# Autodesk Inventor assembly: Frame 1780692296746
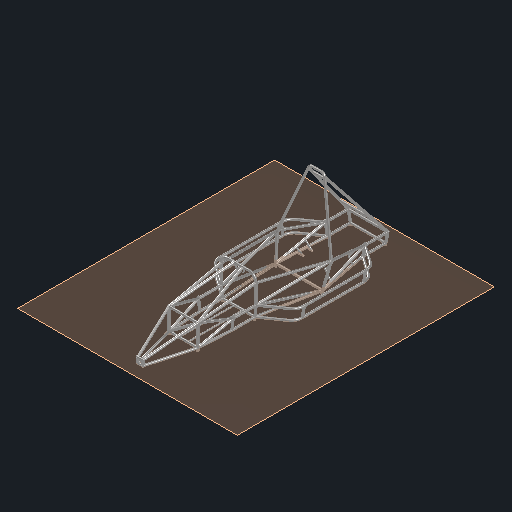
[picture p0: Inventor's stored thumbnail of the model, 512x512]
Saved by Autodesk Inventor 2026.2 (Build 302298010, 298A)
## iProperties
_FrameDoc: Frame Assembly
_Version: 25.0.0
Created: 2026-06-05
Part Number: Frame 1780692296746
Document SubType Name: Assembly
Designer: tasle
Mass: 133713 g
Surface Area: 77277.6 cm^2
Volume: 17033.5 cm^3
Density: 7.85 g/cm^3
Author: tasle
## Documents named in this file (83)
- C:\Users\tasle\Documents\PersonalProjects\FSAE\GOGO_FSAE_CAD\FrameV2\Frame\Frame 1780692296746.iam
- C:\Users\tasle\Documents\PersonalProjects\FSAE\GOGO_FSAE_CAD\FrameV2\Frame\Skeleton 1780692296747.ipt
- C:\Users\tasle\Documents\PersonalProjects\FSAE\GOGO_FSAE_CAD\FrameV2\Frame\ANSI 1 x 0.179 1780692302546.ipt
- C:\Users\tasle\Documents\PersonalProjects\FSAE\GOGO_FSAE_CAD\FrameV2\Frame\ANSI 1 x 0.179 1780692302574.ipt
- C:\Users\tasle\Documents\PersonalProjects\FSAE\GOGO_FSAE_CAD\FrameV2\Frame\ANSI 1 x 0.179 1780692302595.ipt
- C:\Users\tasle\Documents\PersonalProjects\FSAE\GOGO_FSAE_CAD\FrameV2\Frame\ANSI 1 x 0.179 1780692302622.ipt
- C:\Users\tasle\Documents\PersonalProjects\FSAE\GOGO_FSAE_CAD\FrameV2\Frame\ANSI 1 x 0.179 1780692302650.ipt
- C:\Users\tasle\Documents\PersonalProjects\FSAE\GOGO_FSAE_CAD\FrameV2\Frame\ANSI 1 x 0.179 1780692302672.ipt
- C:\Users\tasle\Documents\PersonalProjects\FSAE\GOGO_FSAE_CAD\FrameV2\Frame\ANSI 1 x 0.179 1780692302694.ipt
- C:\Users\tasle\Documents\PersonalProjects\FSAE\GOGO_FSAE_CAD\FrameV2\Frame\ANSI 1 x 0.179 1780692302716.ipt
- C:\Users\tasle\Documents\PersonalProjects\FSAE\GOGO_FSAE_CAD\FrameV2\Frame\ANSI 1 x 0.179 1780692302739.ipt
- C:\Users\tasle\Documents\PersonalProjects\FSAE\GOGO_FSAE_CAD\FrameV2\Frame\ANSI 1 x 0.179 1780692302759.ipt
- C:\Users\tasle\Documents\PersonalProjects\FSAE\GOGO_FSAE_CAD\FrameV2\Frame\ANSI 1 x 0.179 1780692302779.ipt
- C:\Users\tasle\Documents\PersonalProjects\FSAE\GOGO_FSAE_CAD\FrameV2\Frame\ANSI 1 x 0.179 1780692302799.ipt
- C:\Users\tasle\Documents\PersonalProjects\FSAE\GOGO_FSAE_CAD\FrameV2\Frame\ANSI 1 x 0.179 1780692302820.ipt
- C:\Users\tasle\Documents\PersonalProjects\FSAE\GOGO_FSAE_CAD\FrameV2\Frame\ANSI 1 x 0.179 1780692302840.ipt
- C:\Users\tasle\Documents\PersonalProjects\FSAE\GOGO_FSAE_CAD\FrameV2\Frame\ANSI 1 x 0.179 1780692302880.ipt
- C:\Users\tasle\Documents\PersonalProjects\FSAE\GOGO_FSAE_CAD\FrameV2\Frame\ANSI 1 x 0.179 1780692302901.ipt
- C:\Users\tasle\Documents\PersonalProjects\FSAE\GOGO_FSAE_CAD\FrameV2\Frame\ANSI 1 x 0.179 1780692302942.ipt
- C:\Users\tasle\Documents\PersonalProjects\FSAE\GOGO_FSAE_CAD\FrameV2\Frame\ANSI 1 x 0.179 1780692302962.ipt
- C:\Users\tasle\Documents\PersonalProjects\FSAE\GOGO_FSAE_CAD\FrameV2\Frame\ANSI 1 x 0.179 1780692302983.ipt
- C:\Users\tasle\Documents\PersonalProjects\FSAE\GOGO_FSAE_CAD\FrameV2\Frame\ANSI 1 x 0.179 1780692303004.ipt
- C:\Users\tasle\Documents\PersonalProjects\FSAE\GOGO_FSAE_CAD\FrameV2\Frame\ANSI 1 x 0.179 1780692303025.ipt
- C:\Users\tasle\Documents\PersonalProjects\FSAE\GOGO_FSAE_CAD\FrameV2\Frame\ANSI 1 x 0.179 1780692303065.ipt
- C:\Users\tasle\Documents\PersonalProjects\FSAE\GOGO_FSAE_CAD\FrameV2\Frame\ANSI 1 x 0.179 1780692303109.ipt
- C:\Users\tasle\Documents\PersonalProjects\FSAE\GOGO_FSAE_CAD\FrameV2\Frame\ANSI 1 x 0.179 1780692303131.ipt
- C:\Users\tasle\Documents\PersonalProjects\FSAE\GOGO_FSAE_CAD\FrameV2\Frame\ANSI 1 x 0.179 1780692303282.ipt
- C:\Users\tasle\Documents\PersonalProjects\FSAE\GOGO_FSAE_CAD\FrameV2\Frame\ANSI 1 x 0.179 1780692303302.ipt
- C:\Users\tasle\Documents\PersonalProjects\FSAE\GOGO_FSAE_CAD\FrameV2\Frame\ANSI 1 x 0.179 1780692303344.ipt
- C:\Users\tasle\Documents\PersonalProjects\FSAE\GOGO_FSAE_CAD\FrameV2\Frame\ANSI 1 x 0.179 1780692303426.ipt
- C:\Users\tasle\Documents\PersonalProjects\FSAE\GOGO_FSAE_CAD\FrameV2\Frame\ANSI 1 x 0.179 1780692303471.ipt
- C:\Users\tasle\Documents\PersonalProjects\FSAE\GOGO_FSAE_CAD\FrameV2\Frame\ANSI 1 x 0.179 1780692303492.ipt
- C:\Users\tasle\Documents\PersonalProjects\FSAE\GOGO_FSAE_CAD\FrameV2\Frame\ANSI 1 x 0.179 1780692303687.ipt
- C:\Users\tasle\Documents\PersonalProjects\FSAE\GOGO_FSAE_CAD\FrameV2\Frame\ANSI 1 x 0.179 1780692303707.ipt
- C:\Users\tasle\Documents\PersonalProjects\FSAE\GOGO_FSAE_CAD\FrameV2\Frame\ANSI 1 x 0.179 1780692303816.ipt
- C:\Users\tasle\Documents\PersonalProjects\FSAE\GOGO_FSAE_CAD\FrameV2\Frame\ANSI 1 x 0.179 1780692303838.ipt
- C:\Users\tasle\Documents\PersonalProjects\FSAE\GOGO_FSAE_CAD\FrameV2\Frame\ANSI 1 x 0.179 1780692303858.ipt
- C:\Users\tasle\Documents\PersonalProjects\FSAE\GOGO_FSAE_CAD\FrameV2\Frame\ANSI 1 x 0.179 1780692303879.ipt
- C:\Users\tasle\Documents\PersonalProjects\FSAE\GOGO_FSAE_CAD\FrameV2\Frame\ANSI 1 x 0.179 1780692303920.ipt
- C:\Users\tasle\Documents\PersonalProjects\FSAE\GOGO_FSAE_CAD\FrameV2\Frame\ANSI 1 x 0.179 1780692303940.ipt
- C:\Users\tasle\Documents\PersonalProjects\FSAE\GOGO_FSAE_CAD\FrameV2\Frame\ANSI 1 x 0.179 1780692303966.ipt
- C:\Users\tasle\Documents\PersonalProjects\FSAE\GOGO_FSAE_CAD\FrameV2\Frame\ANSI 1 x 0.179 1780692304008.ipt
- C:\Users\tasle\Documents\PersonalProjects\FSAE\GOGO_FSAE_CAD\FrameV2\Frame\ANSI 1 x 0.179 1780692304091.ipt
- C:\Users\tasle\Documents\PersonalProjects\FSAE\GOGO_FSAE_CAD\FrameV2\Frame\ANSI 1 x 0.179 1780692304111.ipt
- C:\Users\tasle\Documents\PersonalProjects\FSAE\GOGO_FSAE_CAD\FrameV2\Frame\ANSI 1 x 0.179 1780692304131.ipt
- C:\Users\tasle\Documents\PersonalProjects\FSAE\GOGO_FSAE_CAD\FrameV2\Frame\ANSI 1 x 0.179 1780692304151.ipt
- C:\Users\tasle\Documents\PersonalProjects\FSAE\GOGO_FSAE_CAD\FrameV2\Frame\ANSI 1 x 0.179 1780692304297.ipt
- C:\Users\tasle\Documents\PersonalProjects\FSAE\GOGO_FSAE_CAD\FrameV2\Frame\ANSI 1 x 0.179 1780692304340.ipt
- C:\Users\tasle\Documents\PersonalProjects\FSAE\GOGO_FSAE_CAD\FrameV2\Frame\ANSI 1 x 0.179 1780692304362.ipt
- C:\Users\tasle\Documents\PersonalProjects\FSAE\GOGO_FSAE_CAD\FrameV2\Frame\ANSI 1 x 0.179 1780692304384.ipt
- C:\Users\tasle\Documents\PersonalProjects\FSAE\GOGO_FSAE_CAD\FrameV2\Frame\ANSI 1 x 0.179 1780692304405.ipt
- C:\Users\tasle\Documents\PersonalProjects\FSAE\GOGO_FSAE_CAD\FrameV2\Frame\ANSI 1 x 0.179 1780692304425.ipt
- C:\Users\tasle\Documents\PersonalProjects\FSAE\GOGO_FSAE_CAD\FrameV2\Frame\ANSI 1 x 0.179 1780692304445.ipt
- C:\Users\tasle\Documents\PersonalProjects\FSAE\GOGO_FSAE_CAD\FrameV2\Frame\ANSI 1 x 0.179 1780692304465.ipt
- C:\Users\tasle\Documents\PersonalProjects\FSAE\GOGO_FSAE_CAD\FrameV2\Frame\ANSI 1 x 0.179 1780692304485.ipt
- C:\Users\tasle\Documents\PersonalProjects\FSAE\GOGO_FSAE_CAD\FrameV2\Frame\ANSI 1 x 0.179 1780692304506.ipt
- C:\Users\tasle\Documents\PersonalProjects\FSAE\GOGO_FSAE_CAD\FrameV2\Frame\ANSI 1 x 0.179 1780692304526.ipt
- C:\Users\tasle\Documents\PersonalProjects\FSAE\GOGO_FSAE_CAD\FrameV2\Frame\ANSI 1 x 0.179 1780692304546.ipt
- C:\Users\tasle\Documents\PersonalProjects\FSAE\GOGO_FSAE_CAD\FrameV2\Frame\ANSI 1 x 0.179 1780692304587.ipt
- C:\Users\tasle\Documents\PersonalProjects\FSAE\GOGO_FSAE_CAD\FrameV2\Frame\ANSI 1 x 0.179 1782332076807.ipt
- C:\Users\tasle\Documents\PersonalProjects\FSAE\GOGO_FSAE_CAD\FrameV2\Frame\ANSI 1 x 0.179 1782332200115.ipt
- C:\Users\tasle\Documents\PersonalProjects\FSAE\GOGO_FSAE_CAD\FrameV2\Frame\ANSI 1 x 0.179 1782332294883.ipt
- C:\Users\tasle\Documents\PersonalProjects\FSAE\GOGO_FSAE_CAD\FrameV2\Frame\ANSI 1 x 0.179 1782332350122.ipt
- C:\Users\tasle\Documents\PersonalProjects\FSAE\GOGO_FSAE_CAD\FrameV2\Frame\ANSI 1 x 0.179 1782332425793.ipt
- C:\Users\tasle\Documents\PersonalProjects\FSAE\GOGO_FSAE_CAD\FrameV2\Frame\ANSI 1 x 0.179 1782332467531.ipt
- C:\Users\tasle\Documents\PersonalProjects\FSAE\GOGO_FSAE_CAD\FrameV2\Frame\ANSI 1 x 0.179 1782334188549.ipt
- C:\Users\tasle\Documents\PersonalProjects\FSAE\GOGO_FSAE_CAD\FrameV2\Frame\ANSI 1 x 0.179 1782334250193.ipt
- C:\Users\tasle\Documents\PersonalProjects\FSAE\GOGO_FSAE_CAD\FrameV2\Frame\ANSI 1_2 x 0.109 1783344969371.ipt
- C:\Users\tasle\Documents\PersonalProjects\FSAE\GOGO_FSAE_CAD\FrameV2\Frame\ANSI 1_2 x 0.109 1783344969395.ipt
- C:\Users\tasle\Documents\PersonalProjects\FSAE\GOGO_FSAE_CAD\FrameV2\Frame\ANSI 1_2 x 0.109 1783352366176.ipt
- C:\Users\tasle\Documents\PersonalProjects\FSAE\GOGO_FSAE_CAD\FrameV2\Frame\ANSI 1_2 x 0.109 1783352366199.ipt
- C:\Users\tasle\Documents\PersonalProjects\FSAE\GOGO_FSAE_CAD\Frame Assembly\FrameV2\Frame\ANSI 1_2 x 0.109 1785174968284.ipt
- C:\Users\tasle\Documents\PersonalProjects\FSAE\GOGO_FSAE_CAD\Frame Assembly\FrameV2\Frame\ANSI 1_2 x 0.109 1785174968323.ipt
- C:\Users\tasle\Documents\PersonalProjects\FSAE\GOGO_FSAE_CAD\Frame Assembly\FrameV2\Frame\ANSI 1_2 x 0.109 1785174968359.ipt
- C:\Users\tasle\Documents\PersonalProjects\FSAE\GOGO_FSAE_CAD\Frame Assembly\FrameV2\Frame\ANSI 1_2 x 0.109 1785177095365.ipt
- C:\Users\tasle\Documents\PersonalProjects\FSAE\GOGO_FSAE_CAD\Frame Assembly\FrameV2\Frame\ANSI 1_2 x 0.109 1785177095400.ipt
- C:\Users\tasle\Documents\PersonalProjects\FSAE\GOGO_FSAE_CAD\Frame Assembly\FrameV2\Frame\ANSI 1_2 x 0.109 1785177095431.ipt
- C:\Users\tasle\Documents\PersonalProjects\FSAE\GOGO_FSAE_CAD\Frame Assembly\FrameV2\Frame\ANSI 1_2 x 0.109 1785264200197.ipt
- C:\Users\tasle\Documents\PersonalProjects\FSAE\GOGO_FSAE_CAD\Frame Assembly\FrameV2\Frame\ANSI 1_2 x 0.109 1785264200234.ipt
- C:\Users\tasle\Documents\PersonalProjects\FSAE\GOGO_FSAE_CAD\Frame Assembly\FrameV2\Frame\ANSI 1_2 x 0.109 1785264200274.ipt
- C:\Users\tasle\Documents\PersonalProjects\FSAE\GOGO_FSAE_CAD\Frame Assembly\FrameV2\Frame\ANSI 1_2 x 0.109 1785264200308.ipt
- C:\Users\tasle\Documents\PersonalProjects\FSAE\GOGO_FSAE_CAD\Frame Assembly\FrameV2\Frame\ANSI 1 x 0.133 1785638103512.ipt
- C:\Users\tasle\Documents\PersonalProjects\FSAE\GOGO_FSAE_CAD\Frame Assembly\FrameV2\Frame\ANSI 1 x 0.133 1785638103546.ipt
## Components (82 placed, 46 different names)
1. Reference Skeleton
2. ANSI 1 x 0.179 - 26.119:1
3. ANSI 1 x 0.179 - 24.499:1
4. ANSI 1 x 0.179 - 26.119:2
5. ANSI 1 x 0.179 - 24.499:2
6. ANSI 1 x 0.179 - 4.076:1
7. ANSI 1 x 0.179 - 4.076:2
8. ANSI 1 x 0.179 - 4.076:3
9. ANSI 1 x 0.179 - 4.076:4
10. ANSI 1 x 0.179 - 15.748:1
11. ANSI 1 x 0.179 - 19.685:1
12. ANSI 1 x 0.179 - 13.971:1
13. ANSI 1 x 0.179 - 17.068:2
14. ANSI 1 x 0.179 - 13.971:2
15. ANSI 1 x 0.179 - 18.741:1
16. ANSI 1 x 0.179 - 18.741:2
17. ANSI 1 x 0.179 - 18.741:3
18. ANSI 1 x 0.179 - 6.935:1
19. ANSI 1 x 0.179 - 18.741:4
20. ANSI 1 x 0.179 - 32.006:1
21. ANSI 1 x 0.179 - 30.721:1
22. ANSI 1 x 0.179 - 30.721:2
23. ANSI 1 x 0.179 - 12.598:4
24. ANSI 1 x 0.179 - 6.935:3
25. ANSI 1 x 0.179 - 12.598:5
26. ANSI 1 x 0.179 - 17.717:1
27. ANSI 1 x 0.179 - 36.643:1
28. ANSI 1 x 0.179 - 36.727:1
29. ANSI 1 x 0.179 - 34.146:1
30. ANSI 1 x 0.179 - 33.363:1
31. ANSI 1 x 0.179 - 5.975:5
32. ANSI 1 x 0.179 - 5.975:6
33. ANSI 1 x 0.179 - 5.975:7
34. ANSI 1 x 0.179 - 36.643:2
35. ANSI 1 x 0.179 - 36.727:2
36. ANSI 1 x 0.179 - 34.146:2
37. ANSI 1 x 0.179 - 33.363:2
38. ANSI 1 x 0.179 - 26.472:1
39. ANSI 1 x 0.179 - 25.469:1
40. ANSI 1 x 0.179 - 23.324:1
41. ANSI 1 x 0.179 - 5.975:8
42. ANSI 1 x 0.179 - 8.022:9
43. ANSI 1 x 0.179 - 8.022:10
44. ANSI 1 x 0.179 - 26.472:2
45. ANSI 1 x 0.179 - 23.324:2
46. ANSI 1 x 0.179 - 47.004:1
47. ANSI 1 x 0.179 - 47.004:2
48. ANSI 1 x 0.179 - 12.598:8
49. ANSI 1 x 0.179 - 25.469:2
50. ANSI 1 x 0.179 - 25.591:1
51. ANSI 1 x 0.179 - 12.598:9
52. ANSI 1 x 0.179 - 7.828:11
53. ANSI 1 x 0.179 - 19.291:2
54. ANSI 1 x 0.179 - 23.264:2
55. ANSI 1 x 0.179 - 12.598:10
56. ANSI 1 x 0.179 - 12.598:11
57. ANSI 1 x 0.179 - 7.828:12
58. ANSI 1 x 0.179 - 32.006:1
59. ANSI 1 x 0.179 - 108.156:1
60. ANSI 1 x 0.179 - 59.522:1
61. ANSI 1 x 0.179 - 70.709:1
62. ANSI 1 x 0.179 - 70.709:2
63. ANSI 1 x 0.179 - 70.709:3
64. ANSI 1 x 0.179 - 70.709:4
65. ANSI 1 x 0.179 - 30.342:1
66. ANSI 1 x 0.179 - 30.342:2
67. ANSI 1/2 x 0.109 - 29.297:1
68. ANSI 1/2 x 0.109 - 29.297:2
69. ANSI 1/2 x 0.109 - 3.643:1
70. ANSI 1/2 x 0.109 - 3.643:2
71. ANSI 1/2 x 0.109 - 9.374:1
72. ANSI 1/2 x 0.109 - 5.512:1
73. ANSI 1/2 x 0.109 - 0.984:1
74. ANSI 1/2 x 0.109 - 5.653:1
75. ANSI 1/2 x 0.109 - 0.787:1
76. ANSI 1/2 x 0.109 - 3.985:1
77. ANSI 1/2 x 0.109 - 4.983:1
78. ANSI 1/2 x 0.109 - 3.937:1
79. ANSI 1/2 x 0.109 - 5.549:1
80. ANSI 1/2 x 0.109 - 3.355:1
81. ANSI 1 x 0.133 - 18.778:1
82. ANSI 1 x 0.133 - 9.836:1
## Relationships (2: Flush 2)
- Flush:1 (1400 mm)
- Flush:2 (200 mm)
